# Autodesk Inventor assembly: undergndPipe
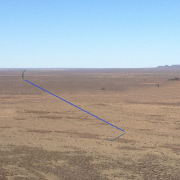
[picture p0: Inventor's stored thumbnail of the model, 180x180]
Saved by Autodesk Inventor 2014 SP1 (Build 180222100, 222)
## iProperties
Created: 2014-03-12
Part Number: undergndPipe
Document SubType Name: Assembly
Designer: Dave
Author: Dave
## Documents named in this file (4)
- C:\Users\Dave\Desktop\hera-cad\Node\undergndPipe.iam
- C:\Users\Dave\Desktop\hera-cad\Node\airgnd_exchange.ipt
- C:\Users\Dave\Desktop\hera-cad\Node\sweep.ipt
- C:\Users\Dave\Desktop\hera-cad\Node\pipe1.5m.ipt
## Components (7 placed, 3 different names)
1. airgnd_exchange:1 — Insert:1, Insert:3, Insert:4
2. sweep:1 — Insert:1, Insert:6
3. sweep:2 — Insert:2
4. sweep:3 — Insert:2, Insert:3
5. sweep:4 — Insert:4, Insert:5
6. sweep:5
7. pipe1.5m:1 — Insert:5, Insert:6
## Relationships (6: Insert 6)
- Insert:1: airgnd_exchange:1 ↔ sweep:1
- Insert:2: sweep:2 ↔ sweep:3
- Insert:3: airgnd_exchange:1 ↔ sweep:3
- Insert:4: airgnd_exchange:1 ↔ sweep:4
- Insert:5: sweep:4 ↔ pipe1.5m:1
- Insert:6: sweep:1 ↔ pipe1.5m:1
